# Autodesk Inventor assembly: Boiler-SubAssy
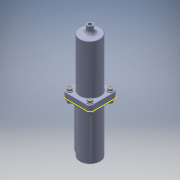
[picture p0: Inventor's stored thumbnail of the model, 180x180]
Saved by Autodesk Inventor 2018 (Build 220112000, 112)
## iProperties
Created: 2020-04-01
Part Number: Boiler-SubAssy
Description: STEP AP214
Document SubType Name: Assembly
Designer: emile
Sending System: SolidWorks 2017
Preprocessor: SwSTEP 2.0
Title: Boiler SubAssy.STEP
Revision Number: ANY
## Documents named in this file (8)
- C:\Users\emile\OneDrive\Documents\GitHub\VentilatorCovid19\Respirator\MultiLine\boiler\Boiler-SubAssy.iam
- C:\Users\emile\OneDrive\Documents\GitHub\VentilatorCovid19\Respirator\MultiLine\boiler\hex flange nut_am_B18.2.2.4M - Hex flange nut, M8 x 1.25 --N.ipt
- C:\Users\emile\OneDrive\Documents\GitHub\VentilatorCovid19\Respirator\MultiLine\boiler\flat washer narrow_am_B18.22M - Plain washer, 8 mm, narrow.ipt
- C:\Users\emile\OneDrive\Documents\GitHub\VentilatorCovid19\Respirator\MultiLine\boiler\formed hex screw_am_B18.2.3.2M - Formed hex screw, M8 x 1.25 x 30 --30WN.ipt
- C:\Users\emile\OneDrive\Documents\GitHub\VentilatorCovid19\Respirator\MultiLine\boiler\Heatting Coil.ipt
- C:\Users\emile\OneDrive\Documents\GitHub\VentilatorCovid19\Respirator\MultiLine\boiler\Boiler Top2.ipt
- C:\Users\emile\OneDrive\Documents\GitHub\VentilatorCovid19\Respirator\MultiLine\boiler\Boiler bottom2.ipt
- C:\Users\emile\OneDrive\Documents\GitHub\VentilatorCovid19\Respirator\MultiLine\boiler\2418T186_ULTRA-COMPRESSIBLE O-RING.ipt
## Components (20 placed, 11 different names)
1. Boiler Top_2 — Mate:2, Mate:6, Mate:7, Mate:8, Mate:9, Flush:1, Flush:2, Mate:10, Mate:11
2. Heatting Coil_20 — Mate:3, Mate:4
3. Boiler bottom2:1 — Mate:2, Mate:3, Mate:4, Mate:5, Tangent:1, Mate:6, Mate:7, Mate:13, Mate:14
4. 2418T186_ULTRA-COMPRESSIBLE O-RING:1 — Mate:5, Tangent:1
5. formed hex screw_am_B18.2.3.2M - Formed hex screw, M8 x 1.25 x 30 --30WN_16 — Mate:10, Mate:12, Mate:17
6. flat washer narrow_am_B18.22M - Plain washer, 8 mm, narrow_10 — Mate:11, Mate:12, Mate:17
7. hex flange nut_am_B18.2.2.4M - Hex flange nut, M8 x 1.25 --N_7 — Mate:15, Mate:16
8. flat washer narrow_am_B18.22M - Plain washer, 8 mm, narrow_9 — Mate:13, Mate:14, Mate:15, Mate:16
9. formed hex screw_am_B18.2.3.2M - Formed hex screw, M8 x 1.25 x 30 --30WN:2
10. flat washer narrow_am_B18.22M - Plain washer, 8 mm, narrow:4
11. hex flange nut_am_B18.2.2.4M - Hex flange nut, M8 x 1.25 --N:5
12. flat washer narrow_am_B18.22M - Plain washer, 8 mm, narrow:5
13. formed hex screw_am_B18.2.3.2M - Formed hex screw, M8 x 1.25 x 30 --30WN:3
14. flat washer narrow_am_B18.22M - Plain washer, 8 mm, narrow:6
15. hex flange nut_am_B18.2.2.4M - Hex flange nut, M8 x 1.25 --N:6
16. flat washer narrow_am_B18.22M - Plain washer, 8 mm, narrow:7
17. formed hex screw_am_B18.2.3.2M - Formed hex screw, M8 x 1.25 x 30 --30WN:4
18. flat washer narrow_am_B18.22M - Plain washer, 8 mm, narrow:8
19. hex flange nut_am_B18.2.2.4M - Hex flange nut, M8 x 1.25 --N:7
20. flat washer narrow_am_B18.22M - Plain washer, 8 mm, narrow:9
## Component patterns: (4 elements, first: formed hex screw_am_B18.2.3.2M - Formed hex screw, M8 x 1.25 x 30 --30WN_16 + flat washer narrow_am_B18.22M - Plain washer, 8 mm, narrow_10 + hex flange nut_am_B18.2.2.4M - Hex flange nut, M8 x 1.25 --N_7 + flat washer narrow_am_B18.22M - Plain washer, 8 mm, narrow_9)
## Relationships (19: Mate 16, Flush 2, Tangent 1)
- Mate:2: Boiler Top_2 ↔ Boiler bottom2:1
- Mate:3: Heatting Coil_20 ↔ Boiler bottom2:1
- Mate:4: Heatting Coil_20 ↔ Boiler bottom2:1
- Mate:5: Boiler bottom2:1 ↔ 2418T186_ULTRA-COMPRESSIBLE O-RING:1
- Tangent:1: Boiler bottom2:1 ↔ 2418T186_ULTRA-COMPRESSIBLE O-RING:1
- Mate:6: Boiler Top_2 ↔ Boiler bottom2:1
- Mate:7: Boiler Top_2 ↔ Boiler bottom2:1
- Mate:8: Boiler Top_2
- Mate:9: Boiler Top_2
- Flush:1: Boiler Top_2
- Flush:2: Boiler Top_2
- Mate:10: Boiler Top_2 ↔ formed hex screw_am_B18.2.3.2M - Formed hex screw, M8 x 1.25 x 30 --30WN_16
- Mate:11: Boiler Top_2 ↔ flat washer narrow_am_B18.22M - Plain washer, 8 mm, narrow_10
- Mate:12: formed hex screw_am_B18.2.3.2M - Formed hex screw, M8 x 1.25 x 30 --30WN_16 ↔ flat washer narrow_am_B18.22M - Plain washer, 8 mm, narrow_10
- Mate:13: Boiler bottom2:1 ↔ flat washer narrow_am_B18.22M - Plain washer, 8 mm, narrow_9
- Mate:14: Boiler bottom2:1 ↔ flat washer narrow_am_B18.22M - Plain washer, 8 mm, narrow_9
- Mate:15: hex flange nut_am_B18.2.2.4M - Hex flange nut, M8 x 1.25 --N_7 ↔ flat washer narrow_am_B18.22M - Plain washer, 8 mm, narrow_9
- Mate:16: hex flange nut_am_B18.2.2.4M - Hex flange nut, M8 x 1.25 --N_7 ↔ flat washer narrow_am_B18.22M - Plain washer, 8 mm, narrow_9
- Mate:17: formed hex screw_am_B18.2.3.2M - Formed hex screw, M8 x 1.25 x 30 --30WN_16 ↔ flat washer narrow_am_B18.22M - Plain washer, 8 mm, narrow_10
